# Autodesk Inventor assembly: Robot
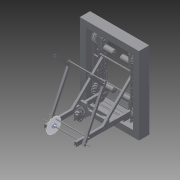
[picture p0: Inventor's stored thumbnail of the model, 180x180]
Saved by Autodesk Inventor 2013 (Build 170138000, 138)
## iProperties
Created: 2014-01-18
Part Number: Robot
Document SubType Name: Assembly
Designer: 272817
Author: 272817
## Documents named in this file (6)
- D:\CAD\2014 Robot\Robot.iam
- D:\CAD\2014 Robot\Frame\Robot Chassis 2014.iam
- D:\CAD\2014 Robot\Bumpers\Bumpers.iam
- D:\CAD\2014 Robot\Ball.ipt
- D:\CAD\2014 Robot\Catapult\Arm\ArmSquare.iam
- D:\CAD\2014 Robot\Catapult\Structure.iam
## Components (5 placed, 5 different names)
1. Robot Chassis 2014:1 [sub-assembly] — Mate:1, Mate:2, Flush:1, Mate:15, Mate:16
2. Bumpers:1 [sub-assembly] — Mate:1, Mate:2, Flush:1, Mate:17
3. Ball:1
4. ArmSquare:2 [sub-assembly] — Mate:18, Mate:19
5. Structure:1 [sub-assembly] — Mate:15, Mate:16, Mate:17, Mate:18, Mate:19
## Relationships (8: Mate 7, Flush 1)
- Mate:1: Robot Chassis 2014:1 ↔ Bumpers:1
- Mate:2 (0.127 mm): Robot Chassis 2014:1 ↔ Bumpers:1
- Flush:1 (30.1625 mm): Robot Chassis 2014:1 ↔ Bumpers:1
- Mate:15: Robot Chassis 2014:1 ↔ Structure:1
- Mate:16: Robot Chassis 2014:1 ↔ Structure:1
- Mate:17 (50.8 mm): Bumpers:1 ↔ Structure:1
- Mate:18: ArmSquare:2 ↔ Structure:1
- Mate:19 (3.175 mm): ArmSquare:2 ↔ Structure:1
